# Autodesk Inventor assembly: Assembly1
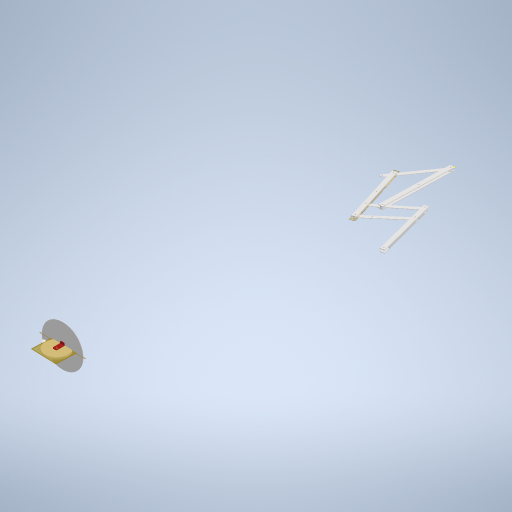
[picture p0: Inventor's stored thumbnail of the model, 512x512]
Saved by Autodesk Inventor 2024 (Build 280153000, 153)
## iProperties
Created: 2024-01-04
Part Number: Assembly1
Document SubType Name: Assembly
Designer: student
Author: student
## Documents named in this file (12)
- D:\TRACER DOCUMENTS\Arm Completed\Assembly1.iam
- D:\TRACER DOCUMENTS\Swerve Drive\ArmBase.ipt
- D:\TRACER DOCUMENTS\Arm\arm gear.iam
- D:\TRACER DOCUMENTS\Swerve Drive\GearSideBracklet.ipt
- D:\TRACER DOCUMENTS\Bracket.ipt
- D:\TRACER DOCUMENTS\Bracket_MIR.ipt
- D:\TRACER DOCUMENTS\Arm\ArmPart1.ipt
- D:\TRACER DOCUMENTS\Arm\ArmPart2.ipt
- D:\TRACER DOCUMENTS\Arm\ArmPart3.ipt
- D:\TRACER DOCUMENTS\Arm\ArmSpacer.ipt
- D:\TRACER DOCUMENTS\Arm\ArmConnector1.ipt
- D:\TRACER DOCUMENTS\Arm\ArmConnector2.ipt
## Components (25 placed, 11 different names)
1. arm gear:1 [sub-assembly] — Mate:2, Mate:3, Flush:2, Flush:3, Flush:4, Flush:5
2. GearSideBracklet:1 — Flush:2, Flush:3, Flush:4, Flush:5
3. ArmBase:1 — Flush:1, Mate:2, Mate:3, Flush:6, Mate:5, Mate:6
4. Bracket:1 — Flush:6, Mate:5, Mate:6
5. <Bracket 2>:1
6. ArmPart1:1 — Mate:7, Mate:9, Mate:10, Mate:13, Mate:18, Mate:19, Mate:50, Mate:51
7. ArmPart2:1 — Mate:46, Mate:47, Mate:48, Mate:49
8. ArmPart3:1 — Mate:52, Mate:53, Mate:54, Mate:55
9. ArmSpacer:1 — Mate:7, Mate:11, Mate:12, Mate:13
10. ArmSpacer:2 — Mate:9, Mate:10
11. ArmConnector1:2 — Mate:11, Mate:12, Mate:20, Mate:21, Mate:22, Mate:23
12. ArmConnector2:1 — Mate:34, Mate:35, Mate:36, Mate:37, Mate:38, Mate:39, Mate:40, Mate:41
13. ArmSpacer:3 — Mate:16, Mate:17, Mate:18, Mate:19
14. ArmSpacer:4 — Mate:14, Mate:15
15. ArmConnector1:3 — Mate:14, Mate:15, Mate:16, Mate:17, Mate:26, Mate:27, Mate:28, Mate:29, Mate:42, Mate:43, Mate:44, Mate:45
16. ArmSpacer:5 — Mate:28, Mate:29, Mate:52, Mate:55
17. ArmSpacer:6 — Mate:20, Mate:21, Mate:53, Mate:54
18. ArmSpacer:7 — Mate:44, Mate:45, Mate:46, Mate:47
19. ArmSpacer:8 — Mate:36, Mate:37
20. ArmSpacer:9 — Mate:22, Mate:23
21. ArmSpacer:10 — Mate:26, Mate:27
22. ArmSpacer:11 — Mate:34, Mate:35, Mate:48, Mate:49
23. ArmSpacer:12 — Mate:38, Mate:39
24. ArmSpacer:13 — Mate:42, Mate:43
25. ArmSpacer:14 — Mate:40, Mate:41, Mate:50, Mate:51
## Relationships (52: Mate 46, Flush 6)
- Flush:1: ArmBase:1
- Mate:2: arm gear:1 ↔ ArmBase:1
- Mate:3 (38.1 mm): arm gear:1 ↔ ArmBase:1
- Flush:2: arm gear:1 ↔ GearSideBracklet:1
- Flush:3: arm gear:1 ↔ GearSideBracklet:1
- Flush:4: arm gear:1 ↔ GearSideBracklet:1
- Flush:5: arm gear:1 ↔ GearSideBracklet:1
- Flush:6: ArmBase:1 ↔ Bracket:1
- Mate:5: ArmBase:1 ↔ Bracket:1
- Mate:6: ArmBase:1 ↔ Bracket:1
- Mate:7: ArmPart1:1 ↔ ArmSpacer:1
- Mate:9: ArmPart1:1 ↔ ArmSpacer:2
- Mate:10: ArmPart1:1 ↔ ArmSpacer:2
- Mate:11: ArmSpacer:1 ↔ ArmConnector1:2
- Mate:12: ArmSpacer:1 ↔ ArmConnector1:2
- Mate:13: ArmPart1:1 ↔ ArmSpacer:1
- Mate:14: ArmSpacer:4 ↔ ArmConnector1:3
- Mate:15: ArmSpacer:4 ↔ ArmConnector1:3
- Mate:16: ArmSpacer:3 ↔ ArmConnector1:3
- Mate:17: ArmSpacer:3 ↔ ArmConnector1:3
- Mate:18: ArmPart1:1 ↔ ArmSpacer:3
- Mate:19: ArmPart1:1 ↔ ArmSpacer:3
- Mate:20: ArmConnector1:2 ↔ ArmSpacer:6
- Mate:21: ArmConnector1:2 ↔ ArmSpacer:6
- Mate:22: ArmConnector1:2 ↔ ArmSpacer:9
- Mate:23: ArmConnector1:2 ↔ ArmSpacer:9
- Mate:26: ArmConnector1:3 ↔ ArmSpacer:10
- Mate:27: ArmConnector1:3 ↔ ArmSpacer:10
- Mate:28: ArmConnector1:3 ↔ ArmSpacer:5
- Mate:29: ArmConnector1:3 ↔ ArmSpacer:5
- Mate:34: ArmConnector2:1 ↔ ArmSpacer:11
- Mate:35: ArmConnector2:1 ↔ ArmSpacer:11
- Mate:36: ArmConnector2:1 ↔ ArmSpacer:8
- Mate:37: ArmConnector2:1 ↔ ArmSpacer:8
- Mate:38: ArmConnector2:1 ↔ ArmSpacer:12
- Mate:39: ArmConnector2:1 ↔ ArmSpacer:12
- Mate:40: ArmConnector2:1 ↔ ArmSpacer:14
- Mate:41: ArmConnector2:1 ↔ ArmSpacer:14
- Mate:42: ArmConnector1:3 ↔ ArmSpacer:13
- Mate:43: ArmConnector1:3 ↔ ArmSpacer:13
- Mate:44: ArmConnector1:3 ↔ ArmSpacer:7
- Mate:45: ArmConnector1:3 ↔ ArmSpacer:7
- Mate:46: ArmPart2:1 ↔ ArmSpacer:7
- Mate:47: ArmPart2:1 ↔ ArmSpacer:7
- Mate:48: ArmPart2:1 ↔ ArmSpacer:11
- Mate:49: ArmPart2:1 ↔ ArmSpacer:11
- Mate:50: ArmPart1:1 ↔ ArmSpacer:14
- Mate:51: ArmPart1:1 ↔ ArmSpacer:14
- Mate:52: ArmPart3:1 ↔ ArmSpacer:5
- Mate:53: ArmPart3:1 ↔ ArmSpacer:6
- Mate:54: ArmPart3:1 ↔ ArmSpacer:6
- Mate:55: ArmPart3:1 ↔ ArmSpacer:5
